# Autodesk Inventor assembly: 000 Ensamblaje hw_DAA - PCB Lemo
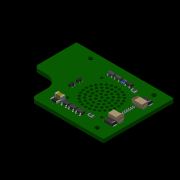
[picture p0: Inventor's stored thumbnail of the model, 180x180]
Saved by Autodesk Inventor 2018 (Build 220112000, 112)
## iProperties
Created: 2024-03-13
Part Number: 000 Ensamblaje hw_DAA - PCB Lemo
Document SubType Name: Assembly
Designer: cda1
Mass: 22.3185 g
Surface Area: 78.0579 cm^2
Volume: 9.84561 cm^3
Density: 2.26685 g/cm^3
Author: cda1
## Documents named in this file (13)
- C:\Users\cda1\Git\DAA\items\hw_DAA\variants\BASIC\3d\000 Ensamblaje hw_DAA - PCB Lemo.iam
- C:\Users\cda1\Git\DAA\items\hw_DAA\3d\hw_DAA - PCB Lemo.ipt
- C:\Users\cda1\Git\DAA\items\_accessories\Componentes PCB\Diodos\3d_Vishay\3d\GSOT05C-HE3-08.ipt
- C:\Users\cda1\Git\DAA\items\_accessories\Componentes PCB\ESD Supressor\3d_Nexperia\PESD15VL2BT-QR\PESD15VL2BT-QR.ipt
- C:\Users\cda1\Git\DAA\items\_accessories\Componentes PCB\ESD Protection\3d_Nexperia\3d\PESD2CANFD27V-UX\PESD2CANFD27V-UX.iam
- C:\Users\cda1\Git\DAA\items\_accessories\Componentes PCB\Diodos\3d_Bourns\3d\SMA6J64CA\SMA6J64CA.ipt
- C:\Users\cda1\Git\DAA\items\_accessories\Componentes PCB\Diodos\3d_Littlefuse\3d\SP712-02HTG\SP712-02HTG.iam
- C:\Users\cda1\Git\DAA\items\_accessories\Componentes PCB\Schottky Diodes\3d_STMicroelectronics\3d\STPS5H100AFY\STPS5H100AFY.ipt
- C:\Users\cda1\Git\DAA\items\_accessories\Componentes PCB\Resistencias\3d_Yageo\3d\AC0805FR-070RL.ipt
- C:\Users\cda1\Git\DAA\items\_accessories\Componentes PCB\Capacitadores\3d_Kemet\3d\C1206C102KGRACAUTO\C1206C102KGRACAUTO.ipt
- C:\Users\cda1\Git\DAA\items\_accessories\Componentes PCB\Resistencias\3d_Stackpole Electronics\HVCB1206FKC1M00\HVCB1206FKC1M00.iam
- C:\Users\cda1\Git\DAA\items\_accessories\Componentes PCB\Resistencias\3d_Vishay\3d\CRCW060310R0FKEAHP\CRCW060310R0FKEAHP.ipt
- C:\Users\cda1\Git\DAA\items\_accessories\Componentes PCB\Resistencias\3d_Panasonic\3d\ERJ-2GE0R00X.ipt
## Components (26 placed, 12 different names)
1. hw_DAA - PCB Lemo:1 — Coincidencia:3, Coincidencia:4, Coincidencia:5, Coincidencia:6, Coincidencia:7, Coincidencia:8, Coincidencia:9, Coincidencia:10, Coincidencia:12, Coincidencia:14, Coincidencia:15, Coincidencia:17, Coincidencia:18, Coincidencia:19, Coincidencia:20, Coincidencia:22, Coincidencia:24, Coincidencia:25, Coincidencia:26, Coincidencia:27, Coincidencia:28, Coincidencia:29, Coincidencia:30, Coincidencia:31, Ángulo:1, Ángulo:2, Ángulo:3, Coincidencia:32, Coincidencia:33, Coincidencia:34, Coincidencia:35, Coincidencia:36, Coincidencia:37, Coincidencia:38, Coincidencia:39, Coincidencia:40
2. GSOT05C-HE3-08:1 — Coincidencia:3, Coincidencia:4
3. GSOT05C-HE3-08:2 — Coincidencia:5, Coincidencia:6
4. GSOT05C-HE3-08:3 — Coincidencia:7, Coincidencia:8
5. PESD15VL2BT-QR:1 — Coincidencia:9, Coincidencia:10, Ángulo:3
6. PESD2CANFD27V-UX:2 [sub-assembly] — Coincidencia:12, Coincidencia:14
7. SMA6J64CA:1 — Coincidencia:15, Ángulo:1
8. SP712-02HTG:1 [sub-assembly] — Coincidencia:17, Coincidencia:19
9. SP712-02HTG:2 [sub-assembly] — Coincidencia:18, Coincidencia:20
10. STPS5H100AFY:1 — Coincidencia:22
11. STPS5H100AFY:2 — Coincidencia:24
12. SMA6J64CA:2 — Coincidencia:25, Ángulo:2
13. AC0805FR-070RL:1 — Coincidencia:26
14. C1206C102KGRACAUTO:1 — Coincidencia:27
15. HVCB1206FKC1M00:1 [sub-assembly] — Coincidencia:28
16. CRCW060310R0FKEAHP:1 — Coincidencia:29
17. PESD2CANFD27V-UX:3 [sub-assembly] — Coincidencia:30, Coincidencia:31
18. AC0805FR-070RL:2 — Coincidencia:32
19. ERJ-2GE0R00X:1 — Coincidencia:33
20. ERJ-2GE0R00X:2 — Coincidencia:34
21. ERJ-2GE0R00X:3 — Coincidencia:35
22. ERJ-2GE0R00X:4 — Coincidencia:36
23. ERJ-2GE0R00X:5 — Coincidencia:37
24. ERJ-2GE0R00X:6 — Coincidencia:38
25. ERJ-2GE0R00X:7 — Coincidencia:39
26. ERJ-2GE0R00X:8 — Coincidencia:40
## Relationships (36: Mate 33, Angle 3)
- Coincidencia:3 [Mate]: hw_DAA - PCB Lemo:1 ↔ GSOT05C-HE3-08:1
- Coincidencia:4 [Mate]: hw_DAA - PCB Lemo:1 ↔ GSOT05C-HE3-08:1
- Coincidencia:5 [Mate]: hw_DAA - PCB Lemo:1 ↔ GSOT05C-HE3-08:2
- Coincidencia:6 [Mate]: hw_DAA - PCB Lemo:1 ↔ GSOT05C-HE3-08:2
- Coincidencia:7 [Mate]: hw_DAA - PCB Lemo:1 ↔ GSOT05C-HE3-08:3
- Coincidencia:8 [Mate]: hw_DAA - PCB Lemo:1 ↔ GSOT05C-HE3-08:3
- Coincidencia:9 [Mate]: hw_DAA - PCB Lemo:1 ↔ PESD15VL2BT-QR:1
- Coincidencia:10 [Mate]: hw_DAA - PCB Lemo:1 ↔ PESD15VL2BT-QR:1
- Coincidencia:12 [Mate]: hw_DAA - PCB Lemo:1 ↔ PESD2CANFD27V-UX:2
- Coincidencia:14 [Mate]: hw_DAA - PCB Lemo:1 ↔ PESD2CANFD27V-UX:2
- Coincidencia:15 [Mate]: hw_DAA - PCB Lemo:1 ↔ SMA6J64CA:1
- Coincidencia:17 [Mate]: hw_DAA - PCB Lemo:1 ↔ SP712-02HTG:1
- Coincidencia:18 [Mate]: hw_DAA - PCB Lemo:1 ↔ SP712-02HTG:2
- Coincidencia:19 [Mate]: hw_DAA - PCB Lemo:1 ↔ SP712-02HTG:1
- Coincidencia:20 [Mate]: hw_DAA - PCB Lemo:1 ↔ SP712-02HTG:2
- Coincidencia:22 [Mate]: hw_DAA - PCB Lemo:1 ↔ STPS5H100AFY:1
- Coincidencia:24 [Mate]: hw_DAA - PCB Lemo:1 ↔ STPS5H100AFY:2
- Coincidencia:25 [Mate]: hw_DAA - PCB Lemo:1 ↔ SMA6J64CA:2
- Coincidencia:26 [Mate]: hw_DAA - PCB Lemo:1 ↔ AC0805FR-070RL:1
- Coincidencia:27 [Mate]: hw_DAA - PCB Lemo:1 ↔ C1206C102KGRACAUTO:1
- Coincidencia:28 [Mate]: hw_DAA - PCB Lemo:1 ↔ HVCB1206FKC1M00:1
- Coincidencia:29 [Mate]: hw_DAA - PCB Lemo:1 ↔ CRCW060310R0FKEAHP:1
- Coincidencia:30 [Mate]: hw_DAA - PCB Lemo:1 ↔ PESD2CANFD27V-UX:3
- Coincidencia:31 [Mate]: hw_DAA - PCB Lemo:1 ↔ PESD2CANFD27V-UX:3
- Ángulo:1 [Angle] (90 deg): hw_DAA - PCB Lemo:1 ↔ SMA6J64CA:1
- Ángulo:2 [Angle] (0 deg): hw_DAA - PCB Lemo:1 ↔ SMA6J64CA:2
- Ángulo:3 [Angle] (0 deg): hw_DAA - PCB Lemo:1 ↔ PESD15VL2BT-QR:1
- Coincidencia:32 [Mate]: hw_DAA - PCB Lemo:1 ↔ AC0805FR-070RL:2
- Coincidencia:33 [Mate]: hw_DAA - PCB Lemo:1 ↔ ERJ-2GE0R00X:1
- Coincidencia:34 [Mate]: hw_DAA - PCB Lemo:1 ↔ ERJ-2GE0R00X:2
- Coincidencia:35 [Mate]: hw_DAA - PCB Lemo:1 ↔ ERJ-2GE0R00X:3
- Coincidencia:36 [Mate]: hw_DAA - PCB Lemo:1 ↔ ERJ-2GE0R00X:4
- Coincidencia:37 [Mate]: hw_DAA - PCB Lemo:1 ↔ ERJ-2GE0R00X:5
- Coincidencia:38 [Mate]: hw_DAA - PCB Lemo:1 ↔ ERJ-2GE0R00X:6
- Coincidencia:39 [Mate]: hw_DAA - PCB Lemo:1 ↔ ERJ-2GE0R00X:7
- Coincidencia:40 [Mate]: hw_DAA - PCB Lemo:1 ↔ ERJ-2GE0R00X:8
